# Autodesk Inventor assembly: Tensioner Type 1
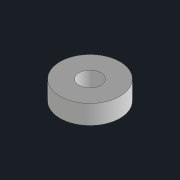
[picture p0: Inventor's stored thumbnail of the model, 180x180]
Saved by Autodesk Inventor 2022 (Build 260153000, 153)
## iProperties
Created: 2022-09-11
Part Number: Tensioner Type 1
Document SubType Name: Assembly
Designer: robpl
Author: robpl
## Documents named in this file (6)
- C:\Users\robpl\OneDrive\Documents\Inventor\2022 FRC Season\Best Coast Drive\Tensioner Type 1.iam
- C:\Users\robpl\OneDrive\Documents\Inventor\2022 FRC Season\Best Coast Drive\5 mm M8 Spacer.ipt
- C:\Users\robpl\OneDrive\Documents\Inventor\2022 FRC Season\Best Coast Drive\22 OD 8ID 7mm Bearing.ipt
- C:\Users\robpl\OneDrive\Documents\Inventor\2022 FRC Season\Best Coast Drive\21.5 mm M8 Spacer.ipt
- C:\Users\robpl\OneDrive\Documents\Inventor\2022 FRC Season\Best Coast Drive\M8 x 50 Button Head Bolt.ipt
- C:\Users\robpl\OneDrive\Documents\Inventor\2022 FRC Season\Best Coast Drive\M8 Nyloc Nut.ipt
## Components (5 placed, 5 different names)
1. 5 mm M8 Spacer:1 — Mate:1, Mate:2, Mate:8
2. 22 OD 8ID 7mm Bearing:1 — Mate:1, Mate:2, Mate:3, Mate:4
3. 21.5 mm M8 Spacer:1 — Mate:3, Mate:4, Mate:5, Mate:6
4. M8 x 50 Button Head Bolt:1 — Mate:5, Mate:6, Mate:7
5. M8 Nyloc Nut:1 — Mate:7, Mate:8
## Relationships (8: Mate 8)
- Mate:1: 5 mm M8 Spacer:1 ↔ 22 OD 8ID 7mm Bearing:1
- Mate:2: 5 mm M8 Spacer:1 ↔ 22 OD 8ID 7mm Bearing:1
- Mate:3: 22 OD 8ID 7mm Bearing:1 ↔ 21.5 mm M8 Spacer:1
- Mate:4: 22 OD 8ID 7mm Bearing:1 ↔ 21.5 mm M8 Spacer:1
- Mate:5: 21.5 mm M8 Spacer:1 ↔ M8 x 50 Button Head Bolt:1
- Mate:6 (3 mm): 21.5 mm M8 Spacer:1 ↔ M8 x 50 Button Head Bolt:1
- Mate:7: M8 x 50 Button Head Bolt:1 ↔ M8 Nyloc Nut:1
- Mate:8 (3 mm): 5 mm M8 Spacer:1 ↔ M8 Nyloc Nut:1
